# Autodesk Inventor assembly: outlets
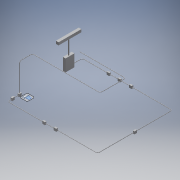
[picture p0: Inventor's stored thumbnail of the model, 180x180]
Saved by Autodesk Inventor 2019 (Build 230136000, 136)
## iProperties
Created: 2018-07-10
Part Number: outlets
Document SubType Name: Assembly
Designer: User
Author: User
## Documents named in this file (12)
- C:\Users\User\Documents\GitHub\darkRadio\3D Models\Room Model\outlets.iam
- C:\Users\User\Documents\GitHub\darkRadio\3D Models\Room Model\outlet.ipt
- C:\Users\User\Documents\GitHub\darkRadio\3D Models\Room Model\left_tube_1.ipt
- C:\Users\User\Documents\GitHub\darkRadio\3D Models\Room Model\leftBack_tube.ipt
- C:\Users\User\Documents\GitHub\darkRadio\3D Models\Room Model\backRight_tube.ipt
- C:\Users\User\Documents\GitHub\darkRadio\3D Models\Room Model\right_tube_0.ipt
- C:\Users\User\Documents\GitHub\darkRadio\3D Models\Room Model\rightFront_tube.ipt
- C:\Users\User\Documents\GitHub\darkRadio\3D Models\Room Model\frontLeft_tube.ipt
- C:\Users\User\Documents\GitHub\darkRadio\3D Models\Room Model\left_tube_0.ipt
- C:\Users\User\Documents\GitHub\darkRadio\3D Models\Room Model\switchbox.ipt
- C:\Users\User\Documents\GitHub\darkRadio\3D Models\Room Model\front_tube_0.ipt
- C:\Users\User\Documents\GitHub\darkRadio\3D Models\Room Model\front_tube_up.ipt
## Components (18 placed, 11 different names)
1. outlet:1 — Rigid:2, Rotational:9, Angle:5
2. left_tube_0:1 — Rigid:2, Rigid:3
3. outlet:2 — Rigid:3, Rigid:4
4. outlet:3 — Rigid:5, Angle:1, Rotational:2, Angle:3
5. left_tube_1:1 — Rigid:4, Rigid:5
6. leftBack_tube:1 — Angle:1, Rotational:2, Rotational:7
7. outlet:4 — Rotational:7, Rotational:3, Angle:2, Angle:3
8. backRight_tube:1 — Rotational:3, Angle:2, Rigid:8
9. outlet:5 — Rigid:8, Rigid:9
10. right_tube_0:1 — Rigid:9, Rigid:10
11. outlet:6 — Rigid:10, Rotational:8, Angle:4
12. rightFront_tube:1 — Rotational:8, Angle:4, Rigid:11
13. outlet:7 — Rigid:11, Flush:1, Rigid:12
14. frontLeft_tube:1 — Rotational:9, Angle:5, Mate:1, Mate:2
15. switchbox:1 — Mate:1, Flush:1, Mate:2
16. front_tube_0:1 — Rigid:12, Rigid:13
17. outlet:8 — Rigid:13, Rotational:15, Angle:6
18. front_tube_up:1 — Rotational:15, Angle:6
## Relationships (25: WeldJoint 10, Angle 6, RevoluteJoint 6, Mate 2, Flush 1)
- Rigid:2 [WeldJoint]: outlet:1 ↔ left_tube_0:1
- Rigid:3 [WeldJoint]: left_tube_0:1 ↔ outlet:2
- Rigid:4 [WeldJoint]: outlet:2 ↔ left_tube_1:1
- Rigid:5 [WeldJoint]: outlet:3 ↔ left_tube_1:1
- Angle:1 (0 deg): outlet:3 ↔ leftBack_tube:1
- Rotational:2 [RevoluteJoint]: outlet:3 ↔ leftBack_tube:1
- Rotational:7 [RevoluteJoint]: leftBack_tube:1 ↔ outlet:4
- Rotational:3 [RevoluteJoint]: outlet:4 ↔ backRight_tube:1
- Angle:2 (0 deg): outlet:4 ↔ backRight_tube:1
- Angle:3 (0 deg): outlet:3 ↔ outlet:4
- Rigid:8 [WeldJoint]: backRight_tube:1 ↔ outlet:5
- Rigid:9 [WeldJoint]: outlet:5 ↔ right_tube_0:1
- Rigid:10 [WeldJoint]: right_tube_0:1 ↔ outlet:6
- Rotational:8 [RevoluteJoint]: outlet:6 ↔ rightFront_tube:1
- Angle:4 (0 deg): outlet:6 ↔ rightFront_tube:1
- Rigid:11 [WeldJoint]: rightFront_tube:1 ↔ outlet:7
- Rotational:9 [RevoluteJoint]: outlet:1 ↔ frontLeft_tube:1
- Angle:5 (0 deg): outlet:1 ↔ frontLeft_tube:1
- Mate:1: frontLeft_tube:1 ↔ switchbox:1
- Flush:1: outlet:7 ↔ switchbox:1
- Mate:2 (-76.2 mm): frontLeft_tube:1 ↔ switchbox:1
- Rigid:12 [WeldJoint]: outlet:7 ↔ front_tube_0:1
- Rigid:13 [WeldJoint]: front_tube_0:1 ↔ outlet:8
- Rotational:15 [RevoluteJoint]: outlet:8 ↔ front_tube_up:1
- Angle:6 (0 deg): outlet:8 ↔ front_tube_up:1
